# Autodesk Inventor assembly: 163321 DNC-32-50-PPV---(asm_0)_CPY
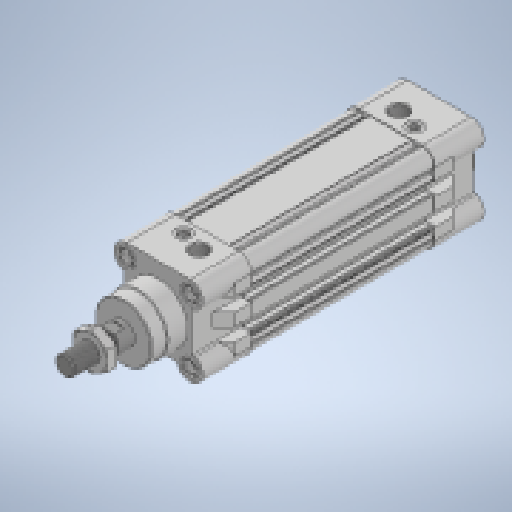
[picture p0: Inventor's stored thumbnail of the model, 512x512]
Saved by Autodesk Inventor 2023 (Build 270158000, 158)
## iProperties
Category: PARTsolutions
Company: FESTO
Created: 2023-04-07
Part Number: 163321 DNC-32-50-PPV---(asm_0)_CPY
Catalog Web Link: www.cadenas.de
Description: DNC-Standard cylinder
Vendor: FESTO
Document SubType Name: Assembly
Designer: Lenovo
Manufacturer: FESTO
Mass: 667 g
Surface Area: 698.502 cm^2
Volume: 226.921 cm^3
Density: 2.93935 g/cm^3
PSOL_IDENT_0: {$CADENAS_DATA/23d-libs/festo/parts/d/dnc/dnc.prj},219 {VTYP=3D},{STYP=ASSTAB},{NB=163321 DNC-32-50-
PSOL_IDENT_1: PPV---(asm_0)},{LINA=163321 DNC-32-50-PPV},{NN=DNC},{DATE=05.04.2023 09:08:13},{GEOMDATE=08.07.2020
PSOL_IDENT_2: 14:00:20},{VERSION=},{LINEID=30},{WBVAR=HUB,HUBST},{WBNUMERIC=HUB,HUBST}  {NB=163321 DNC-32-50-PPV--
PSOL_IDENT_3: -(asm_0)},{LINA=163321 DNC-32-50-PPV},{KT=DUMMY},{TNR=163321},{TYP=DNC},{KDM=32},{HUBX=standard},{HU
PSOL_IDENT_4: BW=50},{HUB=50},{VAR=PPV},{C180=0},{Q=0},{S2=1},{K2=0},{K3=0},{K5=0},{K7=0},{K8=0},{KP=0},{V=0},{HUB
PSOL_IDENT_5: ST=0},{INFO=},{ZZ=0.1},{AM=22.000},{B=30.000},{D2=12.000},{B1=10.000},{D5=32.500},{D7=M6},{D7N=6.000
PSOL_IDENT_6: },{E=45.000},{EE=G1/8},{EEN=9.728},{J3=5.200},{J4=6.000},{J5=44.500},{KK=M10x1,25},{L2=41.600},{L3=1
PSOL_IDENT_7: 12.8},{L31=62.800},{L4=4.000},{L5=25.100},{L6=16.000},{L7=3.300},{L8=10.000},{RT=M6},{VD=18.000},{WH=
PSOL_IDENT_8: 26.000},{ZB=170},{ZB1=120.000},{NA=13.700},{RE=6.250},{VL2=22.000},{KPT=},{KPN=0},{QT=},{QN=0},{S2T=
PSOL_IDENT_9: },{S2N=1},{ZM=97},{VN=0},{VT=},{CPESIZE=14},{A1=35.000},{A2=500.000},{K1=M10},{K2T=},{K3T=},{K5T=},{
PSOL_IDENT_10: K7T=},{K8T=},{P=PPV},{A=0},{MASSBZR=0.517},{MASSHZR=0.030},{MASSBKS=0.162},{MASSHKS=0.009},{CNSMASSE
PSOL_IDENT_11: XACT=0.667},{PPATH=templates/dnc_std_asmtpl.prj},{EOLDATE=},{IDCODE=DNC-32-50-PPV}
NB: 163321 DNC-32-50-PPV---(asm_0)
NN: DNC
NT: Standard cylinder
NBSYN: $TNR. $TYP.-$KDM.-$HUB.-$VAR.---(asm_$HUBST.)
LINA: 163321 DNC-32-50-PPV
CATALOG: Festo
OFFICIAL_STANDARD_NUMBERS: ISO 15552
TNR: 163321
TYP: DNC
KDM: 32
HUB: 50
VAR: PPV
HUBST: 0
AM: 22
B: 30
D2: 12
B1: 10
D5: 32.5
D7: M6
E: 45
EE: G1/8
J3: 5.2
J4: 6
J5: 44.5
KK: M10x1,25
L2: 41.6
L3: 112.8
L4: 4
L5: 25.1
L6: 16
L7: 3.3
L8: 10
RT: M6
VD: 18
WH: 26
ZB: 170
CNSMASSEXACT: 0.667
SUPPLIER: FESTO
ARTICLENO: 163321 DNC-32-50-PPV---(asm_0)
BOMINFO: 163321 DNC-32-50-PPV
CREATOR: CADENAS GmbH
Title: 163321 DNC-32-50-PPV
Author: Cadenas PARTsolutions
Comments: Standard cylinder
## Documents named in this file (4)
- D:\Esdek\Gemelo Digital\Corte de Tubos\CADimportados\PistónHidráulico\163321 DNC-32-50-PPV---(asm_0)_CPY.iam
- D:\Esdek\Gemelo Digital\Corte de Tubos\CADimportados\PistónHidráulico\163321 DNC-32-50---(ZR)_CPY.ipt
- D:\Esdek\Gemelo Digital\Corte de Tubos\CADimportados\PistónHidráulico\DNC-32-50---(KS)_CPY.ipt
- D:\Esdek\Gemelo Digital\Corte de Tubos\CADimportados\PistónHidráulico\DIN-439-B - M10x1_25(F)_CPY.ipt
## Components (3 placed, 3 different names)
1. 163321 DNC-32-50---(ZR)_CPY:1 — KOLBEN_Z@1 <-> ZYLINDER_Z@2, KOLBEN_XY@1 <-> ZYLINDER_XY@2, KOLBEN_YZ@1 <-> ZYLINDER_YZ@2
2. DNC-32-50---(KS)_CPY:1 — KOLBEN_Z@1 <-> ZYLINDER_Z@2, KOLBEN_XY@1 <-> ZYLINDER_XY@2, NUT1_Z@2 <-> din439b_punkt_Z@3, NUT1_XY@2 <-> din439b_punkt_XY@3, KOLBEN_YZ@1 <-> ZYLINDER_YZ@2, NUT1_YZ@2 <-> din439b_punkt_YZ@3
3. DIN-439-B - M10x1_25(F)_CPY:1 — NUT1_Z@2 <-> din439b_punkt_Z@3, NUT1_XY@2 <-> din439b_punkt_XY@3, NUT1_YZ@2 <-> din439b_punkt_YZ@3
## Relationships (6: Mate 3, Angle 2, Flush 1)
- KOLBEN_Z@1 <-> ZYLINDER_Z@2 [Mate]: 163321 DNC-32-50---(ZR)_CPY:1 ↔ DNC-32-50---(KS)_CPY:1
- KOLBEN_XY@1 <-> ZYLINDER_XY@2 [Flush]: 163321 DNC-32-50---(ZR)_CPY:1 ↔ DNC-32-50---(KS)_CPY:1
- NUT1_Z@2 <-> din439b_punkt_Z@3 [Mate]: DNC-32-50---(KS)_CPY:1 ↔ DIN-439-B - M10x1_25(F)_CPY:1
- NUT1_XY@2 <-> din439b_punkt_XY@3 [Mate]: DNC-32-50---(KS)_CPY:1 ↔ DIN-439-B - M10x1_25(F)_CPY:1
- KOLBEN_YZ@1 <-> ZYLINDER_YZ@2 [Angle] (0 deg): 163321 DNC-32-50---(ZR)_CPY:1 ↔ DNC-32-50---(KS)_CPY:1
- NUT1_YZ@2 <-> din439b_punkt_YZ@3 [Angle] (0 deg): DNC-32-50---(KS)_CPY:1 ↔ DIN-439-B - M10x1_25(F)_CPY:1
